# Autodesk Inventor assembly: bed framehalf
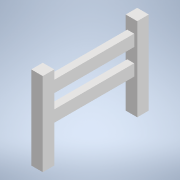
[picture p0: Inventor's stored thumbnail of the model, 180x180]
Saved by Autodesk Inventor 2022 (Build 260153000, 153)
## iProperties
Created: 2022-04-19
Part Number: bed framehalf
Document SubType Name: Assembly
Designer: compsci
Author: compsci
## Documents named in this file (3)
- C:\Users\compsci\Documents\VirtualPeddie\kayebed\bed framehalf.iam
- C:\Users\compsci\Documents\VirtualPeddie\kayebed\column.ipt
- C:\Users\compsci\Documents\VirtualPeddie\kayebed\bar.ipt
## Components (4 placed, 2 different names)
1. column:1 — Mate:1, Mate:2, Flush:2
2. bar:1 — Mate:2, Flush:1, Mate:4
3. bar:2 — Mate:1, Flush:1, Mate:3
4. column:2 — Mate:3, Mate:4, Flush:2
## Relationships (6: Mate 4, Flush 2)
- Mate:1: column:1 ↔ bar:2
- Mate:2: column:1 ↔ bar:1
- Flush:1: bar:1 ↔ bar:2
- Mate:3: bar:2 ↔ column:2
- Mate:4: bar:1 ↔ column:2
- Flush:2: column:1 ↔ column:2
